# Autodesk Inventor assembly: gripper_testing
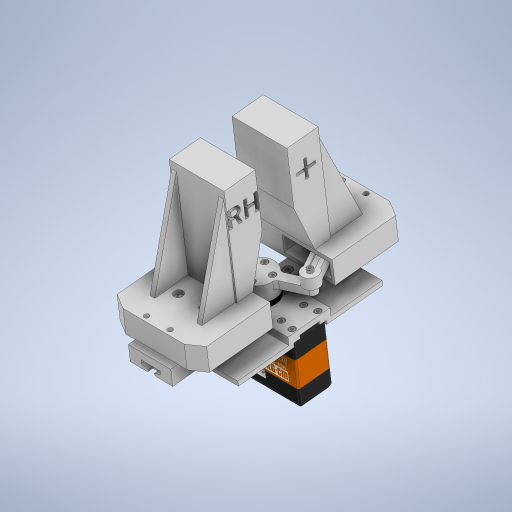
[picture p0: Inventor's stored thumbnail of the model, 512x512]
Saved by Autodesk Inventor 2024 (Build 280153000, 153)
## iProperties
Created: 2023-10-13
Part Number: gripper_testing
Document SubType Name: Assembly
Designer: 박동준
Author: 박동준
## Documents named in this file (11)
- C:\Users\박동준\OneDrive - 연세대학교 (Yonsei University)\바탕 화면\박동준\대학생할\로봇\Humanoid\6축 매니퓰레이터\하드웨어\gripper_testing.iam
- C:\Users\박동준\OneDrive - 연세대학교 (Yonsei University)\바탕 화면\박동준\대학생할\로봇\Humanoid\6축 매니퓰레이터\하드웨어\gripper.ipt
- C:\Users\박동준\OneDrive - 연세대학교 (Yonsei University)\바탕 화면\박동준\대학생할\로봇\Humanoid\6축 매니퓰레이터\하드웨어\gripper_base_frame.ipt
- C:\Users\박동준\OneDrive - 연세대학교 (Yonsei University)\바탕 화면\박동준\대학생할\로봇\Humanoid\6축 매니퓰레이터\하드웨어\axis_7_top_frame.ipt
- C:\Users\박동준\OneDrive - 연세대학교 (Yonsei University)\바탕 화면\박동준\대학생할\로봇\Humanoid\6축 매니퓰레이터\하드웨어\gripper_hand_connector.ipt
- C:\Users\박동준\OneDrive - 연세대학교 (Yonsei University)\바탕 화면\박동준\대학생할\로봇\Humanoid\6축 매니퓰레이터\하드웨어\lm_guide_cart.ipt
- C:\Users\박동준\OneDrive - 연세대학교 (Yonsei University)\바탕 화면\박동준\대학생할\로봇\Humanoid\6축 매니퓰레이터\하드웨어\lm_guide_rail.ipt
- C:\Users\박동준\OneDrive - 연세대학교 (Yonsei University)\바탕 화면\박동준\대학생할\로봇\Humanoid\6축 매니퓰레이터\하드웨어\rh_plus_7_axis_robot_arm_hardware\Part\HTD-45H, Horn\HTD-45H\HTD-45H.iam
- C:\Users\박동준\OneDrive - 연세대학교 (Yonsei University)\바탕 화면\박동준\대학생할\로봇\Humanoid\6축 매니퓰레이터\하드웨어\rh_plus_7_axis_robot_arm_hardware\Part\HTD-45H, Horn\Horn\Top Horn.ipt
- C:\Users\박동준\OneDrive - 연세대학교 (Yonsei University)\바탕 화면\박동준\대학생할\로봇\Humanoid\6축 매니퓰레이터\하드웨어\m2x10.ipt
- C:\Users\박동준\OneDrive - 연세대학교 (Yonsei University)\바탕 화면\박동준\대학생할\로봇\Humanoid\6축 매니퓰레이터\하드웨어\m3x12.ipt
## Components (30 placed, 10 different names)
1. gripper:1 — Mate:22, Mate:23, Angle:4, Flush:1, Mate:44
2. gripper_base_frame:1 — Mate:3, Mate:4, Mate:5, Mate:24, Mate:25, Mate:30, Rotational:1, Rotational:2, Rotational:3, Rotational:4, Mate:43
3. axis_7_top_frame:1 — Mate:10, Mate:11, Angle:1, Mate:12, Mate:13, Mate:14, Mate:15, Mate:16, Mate:17, Rotational:5, Rotational:6, Rotational:7, Rotational:8, Rotational:9, Rotational:10, Rotational:11, Rotational:12
4. gripper_hand_connector:1 — Mate:29, Mate:30, Mate:43, Mate:47, Mate:48
5. lm_guide_cart:1 — Mate:18, Angle:2, Mate:19, Mate:26, Mate:27, Angle:5, Mate:28
6. lm_guide_rail:1 — Mate:12, Mate:13, Mate:14, Mate:18, Angle:2, Mate:19, Rotational:13, Rotational:14
7. HTD-45H:1 [sub-assembly] — Mate:1, Mate:2, Mate:10, Mate:11, Angle:1
8. Top Horn:1 — Mate:1, Mate:2, Mate:3, Mate:4, Mate:5
9. gripper_hand_connector:2 — Mate:22, Mate:23, Mate:24, Mate:25, Mate:45, Mate:46
10. gripper:2 — Mate:26, Mate:27, Angle:5, Mate:28, Mate:29, Flush:1
11. lm_guide_rail:2 — Mate:15, Mate:16, Mate:17, Mate:20, Angle:3, Mate:21, Rotational:15, Rotational:16
12. lm_guide_cart:2 — Mate:20, Angle:3, Mate:21, Angle:4, Mate:44
13. m2x10:1 — Rotational:1
14. m3x12:1 — Rotational:13
15. m2x10:2 — Rotational:2
16. m2x10:3 — Rotational:4
17. m2x10:4 — Rotational:3
18. m2x10:5 — Rotational:5
19. m2x10:6 — Rotational:6
20. m2x10:7 — Rotational:7
21. m2x10:8 — Rotational:8
22. m2x10:9 — Rotational:10
23. m2x10:10 — Rotational:9
24. m2x10:11 — Rotational:11
25. m2x10:12 — Rotational:12
26. m3x12:2 — Rotational:14
27. m3x12:3 — Rotational:16
28. m3x12:4 — Rotational:15
29. m2x10:13 — Mate:45, Mate:46
30. m2x10:14 — Mate:47, Mate:48
## Relationships (54: Mate 32, RevoluteJoint 16, Angle 5, Flush 1)
- Mate:1: HTD-45H:1 ↔ Top Horn:1
- Mate:2: HTD-45H:1 ↔ Top Horn:1
- Mate:3: gripper_base_frame:1 ↔ Top Horn:1
- Mate:4: gripper_base_frame:1 ↔ Top Horn:1
- Mate:5: gripper_base_frame:1 ↔ Top Horn:1
- Mate:10: axis_7_top_frame:1 ↔ HTD-45H:1
- Mate:11: axis_7_top_frame:1 ↔ HTD-45H:1
- Angle:1 (0 deg): axis_7_top_frame:1 ↔ HTD-45H:1
- Mate:12: axis_7_top_frame:1 ↔ lm_guide_rail:1
- Mate:13: axis_7_top_frame:1 ↔ lm_guide_rail:1
- Mate:14: axis_7_top_frame:1 ↔ lm_guide_rail:1
- Mate:15: axis_7_top_frame:1 ↔ lm_guide_rail:2
- Mate:16: axis_7_top_frame:1 ↔ lm_guide_rail:2
- Mate:17: axis_7_top_frame:1 ↔ lm_guide_rail:2
- Mate:18: lm_guide_cart:1 ↔ lm_guide_rail:1
- Angle:2 (0 deg): lm_guide_cart:1 ↔ lm_guide_rail:1
- Mate:19: lm_guide_cart:1 ↔ lm_guide_rail:1
- Mate:20: lm_guide_rail:2 ↔ lm_guide_cart:2
- Angle:3 (0 deg): lm_guide_rail:2 ↔ lm_guide_cart:2
- Mate:21: lm_guide_rail:2 ↔ lm_guide_cart:2
- Mate:22: gripper:1 ↔ gripper_hand_connector:2
- Mate:23: gripper:1 ↔ gripper_hand_connector:2
- Mate:24: gripper_base_frame:1 ↔ gripper_hand_connector:2
- Mate:25: gripper_base_frame:1 ↔ gripper_hand_connector:2
- Angle:4 (0 deg): gripper:1 ↔ lm_guide_cart:2
- Mate:26: lm_guide_cart:1 ↔ gripper:2
- Mate:27: lm_guide_cart:1 ↔ gripper:2
- Angle:5 (0 deg): lm_guide_cart:1 ↔ gripper:2
- Mate:28: lm_guide_cart:1 ↔ gripper:2
- Mate:29: gripper_hand_connector:1 ↔ gripper:2
- Mate:30: gripper_base_frame:1 ↔ gripper_hand_connector:1
- Flush:1: gripper:1 ↔ gripper:2
- Rotational:1 [RevoluteJoint]: gripper_base_frame:1 ↔ m2x10:1
- Rotational:2 [RevoluteJoint]: gripper_base_frame:1 ↔ m2x10:2
- Rotational:3 [RevoluteJoint]: gripper_base_frame:1 ↔ m2x10:4
- Rotational:4 [RevoluteJoint]: gripper_base_frame:1 ↔ m2x10:3
- Mate:43: gripper_base_frame:1 ↔ gripper_hand_connector:1
- Rotational:5 [RevoluteJoint]: axis_7_top_frame:1 ↔ m2x10:5
- Rotational:6 [RevoluteJoint]: axis_7_top_frame:1 ↔ m2x10:6
- Rotational:7 [RevoluteJoint]: axis_7_top_frame:1 ↔ m2x10:7
- Rotational:8 [RevoluteJoint]: axis_7_top_frame:1 ↔ m2x10:8
- Rotational:9 [RevoluteJoint]: axis_7_top_frame:1 ↔ m2x10:10
- Rotational:10 [RevoluteJoint]: axis_7_top_frame:1 ↔ m2x10:9
- Rotational:11 [RevoluteJoint]: axis_7_top_frame:1 ↔ m2x10:11
- Rotational:12 [RevoluteJoint]: axis_7_top_frame:1 ↔ m2x10:12
- Rotational:13 [RevoluteJoint]: lm_guide_rail:1 ↔ m3x12:1
- Rotational:14 [RevoluteJoint]: lm_guide_rail:1 ↔ m3x12:2
- Rotational:15 [RevoluteJoint]: lm_guide_rail:2 ↔ m3x12:4
- Mate:44: gripper:1 ↔ lm_guide_cart:2
- Rotational:16 [RevoluteJoint]: lm_guide_rail:2 ↔ m3x12:3
- Mate:45: gripper_hand_connector:2 ↔ m2x10:13
- Mate:46: gripper_hand_connector:2 ↔ m2x10:13
- Mate:47: gripper_hand_connector:1 ↔ m2x10:14
- Mate:48: gripper_hand_connector:1 ↔ m2x10:14
